# Autodesk Inventor assembly: chassisassembly(ca)
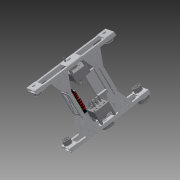
[picture p0: Inventor's stored thumbnail of the model, 180x180]
Saved by Autodesk Inventor 2015 (Build 190159000, 159)
## iProperties
Created: 2015-10-09
Part Number: chassisassembly(ca)
Document SubType Name: Assembly
Designer: elilitwack
Mass: 5923.25 g
Surface Area: 22541.6 cm^2
Volume: 2428.5 cm^3
Density: 2.43906 g/cm^3
RuleStatus: InUse
Author: elilitwack
## Documents named in this file (14)
- C:\Users\elilitwack\Documents\2015 Offseason Chassis\West Coast Chassis Fall 2015 - iLogic\chassisassembly(ca).iam
- C:\Users\elilitwack\Documents\2015 Offseason Chassis\West Coast Chassis Fall 2015 - iLogic\sideassembly(sa).iam
- C:\Users\elilitwack\Documents\2015 Offseason Chassis\West Coast Chassis Fall 2015 - iLogic\crossbar(cb).ipt
- C:\Users\elilitwack\Documents\2015 Offseason Chassis\West Coast Chassis Fall 2015 - iLogic\sideassembly(sa)_MIR.iam
- C:\Users\elilitwack\Documents\2015 Offseason Chassis\West Coast Chassis Fall 2015 - iLogic\Imported Components\217-4244\217-4244.ipt
- C:\Users\elilitwack\Documents\2015 Offseason Chassis\West Coast Chassis Fall 2015 - iLogic\bh_base.ipt
- C:\Users\elilitwack\Documents\2015 Offseason Chassis\West Coast Chassis Fall 2015 - iLogic\cross_structural_plate(csp).ipt
- C:\Users\elilitwack\Documents\2015 Offseason Chassis\West Coast Chassis Fall 2015 - iLogic\standoff(so).ipt
- C:\Users\elilitwack\Documents\2015 Offseason Chassis\West Coast Chassis Fall 2015 - iLogic\Imported Components\supershifter\supershifter.iam
- C:\Users\elilitwack\Documents\2015 Offseason Chassis\West Coast Chassis Fall 2015 - iLogic\Imported Components\39 tooth pulley assembly\39 tooth pulley assembly.iam
- C:\Users\elilitwack\Documents\2015 Offseason Chassis\West Coast Chassis Fall 2015 - iLogic\half_moon(hm).ipt
- C:\Users\elilitwack\Documents\2015 Offseason Chassis\West Coast Chassis Fall 2015 - iLogic\Imported Components\4PlactionWheel-asm\4PlactionWheel-asm.iam
- C:\Users\elilitwack\Documents\2015 Offseason Chassis\West Coast Chassis Fall 2015 - iLogic\Imported Components\am-0145+Updated+Toughbox+2015\am-0145+Updated+Toughbox+2015.iam
- C:\Users\elilitwack\Documents\2015 Offseason Chassis\West Coast Chassis Fall 2015 - iLogic\gearbox(gb).xlsx
## Components (31 placed, 12 different names)
1. sideassembly(sa):1 [sub-assembly] — Mate:1, Mate:2, Mate:3, Mate:4, Mate:5, Mate:6, Mate:7, Mate:8, Mate:9, Mate:10, Mate:11, Mate:12, Mate:42, Mate:43, Mate:44, Mate:45, Mate:46, Mate:47, Mate:48, Mate:49, Mate:72, Mate:73, Mate:85, Mate:89
2. crossbar(cb):1 — Mate:1, Mate:2, Mate:3, Mate:18, Mate:19, Mate:20, Mate:33, Mate:34
3. crossbar(cb):2 — Mate:4, Mate:5, Mate:6, Mate:35, Mate:41
4. crossbar(cb):3 — Mate:10, Mate:11, Mate:12, Mate:13, Mate:14, Mate:15, Mate:36, Mate:38, Mate:40
5. crossbar(cb):4 — Mate:7, Mate:8, Mate:9, Mate:30, Mate:31, Mate:32, Mate:37, Mate:39
6. sideassembly(sa)_MIR:1 [sub-assembly] — Mate:13, Mate:14, Mate:15, Mate:39, Mate:40, Mate:41, Mate:50, Mate:51, Mate:52, Mate:53, Mate:54, Mate:55, Mate:56, Mate:57, Mate:70, Mate:71, Mate:78, Mate:79, Mate:81, Mate:82, Mate:83, Mate:84, Mate:86, Mate:87
7. 217-4244:1 — Mate:18, Mate:19, Mate:20
8. bh_base:1 — Mate:30, Mate:31, Mate:32
9. cross_structural_plate(csp):1 — Mate:33, Mate:34, Mate:35
10. cross_structural_plate(csp):2 — Mate:36, Mate:37, Mate:38
11. standoff(so):1 — Mate:45, Mate:46, Mate:60, Mate:65
12. standoff(so):2 — Mate:44, Mate:48
13. standoff(so):3 — Mate:43, Mate:49
14. standoff(so):4 — Mate:42, Mate:47, Mate:64, Mate:90, Mate:91
15. standoff(so):5 — Mate:53, Mate:54, Mate:63
16. standoff(so):6 — Mate:52, Mate:56
17. standoff(so):7 — Mate:50, Mate:55, Mate:61, Mate:62, Mate:88
18. standoff(so):8 — Mate:51, Mate:57
19. supershifter:1 [sub-assembly] — Mate:61, Mate:62, Mate:63, Mate:68, Mate:76, Mate:77
20. supershifter:2 [sub-assembly] — Mate:60, Mate:64, Mate:65, Mate:69, Mate:74, Mate:75
21. 39 tooth pulley assembly:1 [sub-assembly] — Mate:69, Mate:85
22. 39 tooth pulley assembly:2 [sub-assembly] — Mate:68, Mate:84
23. 39 tooth pulley assembly:3 [sub-assembly] — Mate:72, Mate:75
24. 39 tooth pulley assembly:4 [sub-assembly] — Mate:73, Mate:74
25. 39 tooth pulley assembly:5 [sub-assembly] — Mate:71, Mate:77
26. 39 tooth pulley assembly:6 [sub-assembly] — Mate:70, Mate:76
27. half_moon(hm):1 — Mate:78, Mate:79
28. 4PlactionWheel-asm:1 [sub-assembly] — Mate:82, Mate:83
29. 4PlactionWheel-asm:2 [sub-assembly] — Mate:81
30. toughbox:1 [sub-assembly] — Mate:89, Mate:90, Mate:91
31. toughbox:2 [sub-assembly] — Mate:86, Mate:87, Mate:88
## Relationships (75: Mate 75)
- Mate:1: sideassembly(sa):1 ↔ crossbar(cb):1
- Mate:2: sideassembly(sa):1 ↔ crossbar(cb):1
- Mate:3: sideassembly(sa):1 ↔ crossbar(cb):1
- Mate:4: sideassembly(sa):1 ↔ crossbar(cb):2
- Mate:5: sideassembly(sa):1 ↔ crossbar(cb):2
- Mate:6: sideassembly(sa):1 ↔ crossbar(cb):2
- Mate:7: sideassembly(sa):1 ↔ crossbar(cb):4
- Mate:8: sideassembly(sa):1 ↔ crossbar(cb):4
- Mate:9: sideassembly(sa):1 ↔ crossbar(cb):4
- Mate:10: sideassembly(sa):1 ↔ crossbar(cb):3
- Mate:11: sideassembly(sa):1 ↔ crossbar(cb):3
- Mate:12: sideassembly(sa):1 ↔ crossbar(cb):3
- Mate:13: crossbar(cb):3 ↔ sideassembly(sa)_MIR:1
- Mate:14: crossbar(cb):3 ↔ sideassembly(sa)_MIR:1
- Mate:15: crossbar(cb):3 ↔ sideassembly(sa)_MIR:1
- Mate:18: crossbar(cb):1 ↔ 217-4244:1
- Mate:19: crossbar(cb):1 ↔ 217-4244:1
- Mate:20: crossbar(cb):1 ↔ 217-4244:1
- Mate:30: crossbar(cb):4 ↔ bh_base:1
- Mate:31: crossbar(cb):4 ↔ bh_base:1
- Mate:32: crossbar(cb):4 ↔ bh_base:1
- Mate:33: crossbar(cb):1 ↔ cross_structural_plate(csp):1
- Mate:34: crossbar(cb):1 ↔ cross_structural_plate(csp):1
- Mate:35: crossbar(cb):2 ↔ cross_structural_plate(csp):1
- Mate:36: crossbar(cb):3 ↔ cross_structural_plate(csp):2
- Mate:37: crossbar(cb):4 ↔ cross_structural_plate(csp):2
- Mate:38: crossbar(cb):3 ↔ cross_structural_plate(csp):2
- Mate:39: crossbar(cb):4 ↔ sideassembly(sa)_MIR:1
- Mate:40: crossbar(cb):3 ↔ sideassembly(sa)_MIR:1
- Mate:41: crossbar(cb):2 ↔ sideassembly(sa)_MIR:1
- Mate:42: sideassembly(sa):1 ↔ standoff(so):4
- Mate:43: sideassembly(sa):1 ↔ standoff(so):3
- Mate:44: sideassembly(sa):1 ↔ standoff(so):2
- Mate:45: sideassembly(sa):1 ↔ standoff(so):1
- Mate:46: sideassembly(sa):1 ↔ standoff(so):1
- Mate:47: sideassembly(sa):1 ↔ standoff(so):4
- Mate:48: sideassembly(sa):1 ↔ standoff(so):2
- Mate:49: sideassembly(sa):1 ↔ standoff(so):3
- Mate:50: sideassembly(sa)_MIR:1 ↔ standoff(so):7
- Mate:51: sideassembly(sa)_MIR:1 ↔ standoff(so):8
- Mate:52: sideassembly(sa)_MIR:1 ↔ standoff(so):6
- Mate:53: sideassembly(sa)_MIR:1 ↔ standoff(so):5
- Mate:54: sideassembly(sa)_MIR:1 ↔ standoff(so):5
- Mate:55: sideassembly(sa)_MIR:1 ↔ standoff(so):7
- Mate:56: sideassembly(sa)_MIR:1 ↔ standoff(so):6
- Mate:57: sideassembly(sa)_MIR:1 ↔ standoff(so):8
- Mate:60: standoff(so):1 ↔ supershifter:2
- Mate:61: standoff(so):7 ↔ supershifter:1
- Mate:62: standoff(so):7 ↔ supershifter:1
- Mate:63: standoff(so):5 ↔ supershifter:1
- Mate:64: standoff(so):4 ↔ supershifter:2
- Mate:65: standoff(so):1 ↔ supershifter:2
- Mate:68: supershifter:1 ↔ 39 tooth pulley assembly:2
- Mate:69: supershifter:2 ↔ 39 tooth pulley assembly:1
- Mate:70: sideassembly(sa)_MIR:1 ↔ 39 tooth pulley assembly:6
- Mate:71: sideassembly(sa)_MIR:1 ↔ 39 tooth pulley assembly:5
- Mate:72: sideassembly(sa):1 ↔ 39 tooth pulley assembly:3
- Mate:73: sideassembly(sa):1 ↔ 39 tooth pulley assembly:4
- Mate:74: supershifter:2 ↔ 39 tooth pulley assembly:4
- Mate:75: supershifter:2 ↔ 39 tooth pulley assembly:3
- Mate:76: supershifter:1 ↔ 39 tooth pulley assembly:6
- Mate:77: supershifter:1 ↔ 39 tooth pulley assembly:5
- Mate:78: sideassembly(sa)_MIR:1 ↔ half_moon(hm):1
- Mate:79: sideassembly(sa)_MIR:1 ↔ half_moon(hm):1
- Mate:81: sideassembly(sa)_MIR:1 ↔ 4PlactionWheel-asm:2
- Mate:82: sideassembly(sa)_MIR:1 ↔ 4PlactionWheel-asm:1
- Mate:83: sideassembly(sa)_MIR:1 ↔ 4PlactionWheel-asm:1
- Mate:84: sideassembly(sa)_MIR:1 ↔ 39 tooth pulley assembly:2
- Mate:85: sideassembly(sa):1 ↔ 39 tooth pulley assembly:1
- Mate:86: sideassembly(sa)_MIR:1 ↔ toughbox:2
- Mate:87: sideassembly(sa)_MIR:1 ↔ toughbox:2
- Mate:88: standoff(so):7 ↔ toughbox:2
- Mate:89: sideassembly(sa):1 ↔ toughbox:1
- Mate:90: standoff(so):4 ↔ toughbox:1
- Mate:91: standoff(so):4 ↔ toughbox:1
## Named parameters: gb_mh_seperation = 111.1504 mm, gb_mh_diameter = 6.35 mm, gb_axle_from_edge = 38.1 mm, gb_width = 127 mm, gb_bearing_diameter = 28.575 mm, gb_to_bottom_of_side_assembly = 4.7752 mm, gb_is_ss = 1, gb_mh_seperation_alt = 111.125 mm, gb_axle_from_edge_alt = 43.1546 mm
